# Autodesk Inventor assembly: Hanging Corner Cupboard (concept)
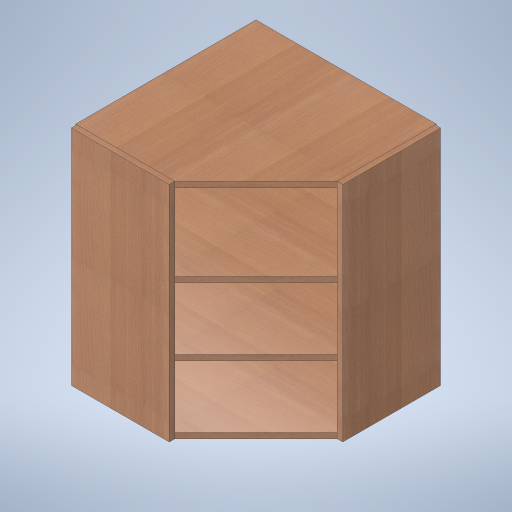
[picture p0: Inventor's stored thumbnail of the model, 512x512]
Saved by Autodesk Inventor 2024 (Build 280153000, 153)
## iProperties
RuleStatus: InUse
Created: 2017-01-19
Part Number: Hanging Corner Cupboard (concept)
Document SubType Name: Assembly
Designer: SvetlanaB
Author: SvetlanaB
## Documents named in this file (16)
- C:\W4INV 2024 Design\iBOX LIBRARY\Kitchen\Wall Cabinets\Corner Cupboard\Corner Cupboard.iam
- C:\W4INV 2024 Design\iBOX LIBRARY\Kitchen\Wall Cabinets\Corner Cupboard\Top.ipt
- C:\W4INV 2024 Design\iBOX LIBRARY\Kitchen\Wall Cabinets\Corner Cupboard\Right_side.ipt
- C:\W4INV 2024 Design\iBOX LIBRARY\Kitchen\Wall Cabinets\Corner Cupboard\Left_side.ipt
- C:\W4INV 2024 Design\iBOX LIBRARY\Kitchen\Wall Cabinets\Corner Cupboard\Back_panel.ipt
- C:\W4INV 2024 Design\iBOX LIBRARY\Kitchen\Wall Cabinets\Corner Cupboard\Back_left_panel.ipt
- C:\W4INV 2024 Design\iBOX LIBRARY\Kitchen\Wall Cabinets\Corner Cupboard\Back_right_panel.ipt
- C:\W4INV 2024 Design\_LIBRARY\Fixed joints\Minifix joint\MINIFIX D15 v2\Minifix D15 & Dowel L34 & Cap D15 PB T18 LH.ipt
- C:\W4INV 2024 Design\_LIBRARY\Fixed joints\Minifix joint\MINIFIX D15 v2\Minifix D15 & Dowel L34 & Cap D15 PB T18 RH.ipt
- C:\W4INV 2024 Design\iBOX LIBRARY\Kitchen\Wall Cabinets\Corner Cupboard\Cupboard (concept).ipt
- C:\W4INV 2024 Design\iBOX LIBRARY\Kitchen\Wall Cabinets\Corner Cupboard\Shelf.ipt
- C:\W4INV 2024 Design\_LIBRARY\Holders\Shelf holder D5\Shelf support D5 L16 with hole covers.ipt
- C:\W4INV 2024 Design\iBOX LIBRARY\Kitchen\Wall Cabinets\Corner Cupboard\Bottom.ipt
- C:\W4INV 2024 Design\_LIBRARY\Fixed joints\Minifix joint\MINIFIX D15 v2\Minifix D15 & Dowel L34 & Cap D15 PB T18 BT.ipt
- C:\W4INV 2023 Design\LIBRARY\Fixed joints\Minifix joint\MINIFIX D15 v2.ipt
- C:\W4INV 2023 Design\LIBRARY\Holders\Shelf holder D5.ipt
## Components (30 placed, 13 different names)
1. @Skeleton
2. Top:1 — Pillar Board Side Plane :1, Pillar Board Side Plane :2, Pillar Board Side Plane :5, Pillar Board Side Plane :6, Nestled Board Plane:9
3. Right_side:1 — Flush:2, Flush:4, Nestled Board Plane:5, Nestled Board Plane:6, Nestled Board Plane:7, Nestled Board Plane:8, Side Board Plane:3, Side Board Plane:4
4. Left_side:1 — Flush:1, Flush:3, Nestled Board Plane:1, Nestled Board Plane:2, Nestled Board Plane:3, Nestled Board Plane:4, Side Board Plane:1, Side Board Plane:2
5. Back_panel:1 — Pillar Board Side Plane :9, Pillar Board Side Plane :10, Side Board Plane:5
6. Back_left_panel:1
7. Back_right_panel:1
8. Minifix D15 & Dowel L34 & Cap D15 PB T18 RH:1 — Axis Plane:1, Nestled Board Plane:1, Pillar Board Side Plane :1
9. Minifix D15 & Dowel L34 & Cap D15 PB T18 LH:2 — Axis Plane:2, Nestled Board Plane:2, Pillar Board Side Plane :2
10. Minifix D15 & Dowel L34 & Cap D15 PB T18 LH:3 — Axis Plane:3, Nestled Board Plane:3, Axis Plane:11, Axis Plane:12, Axis Plane:13, Pillar Board Side Plane :3
11. Minifix D15 & Dowel L34 & Cap D15 PB T18 RH:4 — Axis Plane:4, Nestled Board Plane:4, Axis Plane:14, Pillar Board Side Plane :4
12. Minifix D15 & Dowel L34 & Cap D15 PB T18 LH:5 — Axis Plane:5, Nestled Board Plane:5, Pillar Board Side Plane :5
13. Minifix D15 & Dowel L34 & Cap D15 PB T18 RH:6 — Axis Plane:6, Nestled Board Plane:6, Pillar Board Side Plane :6
14. Minifix D15 & Dowel L34 & Cap D15 PB T18 RH:7 — Axis Plane:7, Nestled Board Plane:7, Pillar Board Side Plane :7
15. Minifix D15 & Dowel L34 & Cap D15 PB T18 LH:8 — Axis Plane:8, Nestled Board Plane:8, Pillar Board Side Plane :8
16. Minifix D15 & Dowel L34 & Cap D15 PB T18 BT:9 — Nestled Board Plane:9, Pillar Board Side Plane :9, Axis Plane:9
17. Minifix D15 & Dowel L34 & Cap D15 PB T18 BT:10 — Pillar Board Side Plane :10, Axis Plane:10, Axis Plane:15, Axis Plane:16, Nestled Board Plane:10
18. Bottom:1 — Nestled Board Plane:10, Pillar Board Side Plane :3, Pillar Board Side Plane :4, Pillar Board Side Plane :7, Pillar Board Side Plane :8
19. Shelf:1 — Shelf Pottom Plane:1, Shelf Pottom Plane:2, Shelf Pottom Plane:3, Shelf Pottom Plane:4, Shelf Pottom Plane:5
20. Shelf support D5 L16 with hole covers:2 — Axis Plane:18, Side Board Plane:2, Shelf Pottom Plane:2
21. Shelf support D5 L16 with hole covers:1 — Axis Plane:17, Side Board Plane:1, Shelf Pottom Plane:1
22. Shelf support D5 L16 with hole covers:5 — Side Board Plane:5, Shelf Pottom Plane:5, Axis Plane:21
23. Shelf support D5 L16 with hole covers:3 — Axis Plane:19, Side Board Plane:3, Shelf Pottom Plane:3
24. Shelf support D5 L16 with hole covers:4 — Axis Plane:20, Side Board Plane:4, Shelf Pottom Plane:4
25. Shelf:2
26. Shelf support D5 L16 with hole covers:6
27. Shelf support D5 L16 with hole covers:7
28. Shelf support D5 L16 with hole covers:8
29. Shelf support D5 L16 with hole covers:9
30. Shelf support D5 L16 with hole covers:10
## Component patterns: (2 elements, first: Shelf:1 + Shelf support D5 L16 with hole covers:2 + Shelf support D5 L16 with hole covers:1 + Shelf support D5 L16 with hole covers:5 + Shelf support D5 L16 with hole covers:3 + Shelf support D5 L16 with hole covers:4)
## Relationships (55: Mate 41, Flush 14)
- Flush:1 (-75 mm): Left_side:1
- Flush:2 (-75 mm): Right_side:1
- Flush:3 (-75 mm): Left_side:1
- Flush:4 (-75 mm): Right_side:1
- Axis Plane:1 [Mate]: Minifix D15 & Dowel L34 & Cap D15 PB T18 RH:1
- Nestled Board Plane:1 [Mate]: Left_side:1 ↔ Minifix D15 & Dowel L34 & Cap D15 PB T18 RH:1
- Pillar Board Side Plane :1 [Flush] (18 mm): Top:1 ↔ Minifix D15 & Dowel L34 & Cap D15 PB T18 RH:1
- Axis Plane:2 [Mate]: Minifix D15 & Dowel L34 & Cap D15 PB T18 LH:2
- Nestled Board Plane:2 [Mate]: Left_side:1 ↔ Minifix D15 & Dowel L34 & Cap D15 PB T18 LH:2
- Pillar Board Side Plane :2 [Flush] (18 mm): Top:1 ↔ Minifix D15 & Dowel L34 & Cap D15 PB T18 LH:2
- Axis Plane:3 [Mate]: Minifix D15 & Dowel L34 & Cap D15 PB T18 LH:3
- Nestled Board Plane:3 [Mate]: Left_side:1 ↔ Minifix D15 & Dowel L34 & Cap D15 PB T18 LH:3
- Axis Plane:4 [Mate]: Minifix D15 & Dowel L34 & Cap D15 PB T18 RH:4
- Nestled Board Plane:4 [Mate]: Left_side:1 ↔ Minifix D15 & Dowel L34 & Cap D15 PB T18 RH:4
- Axis Plane:5 [Mate]: Minifix D15 & Dowel L34 & Cap D15 PB T18 LH:5
- Nestled Board Plane:5 [Mate]: Right_side:1 ↔ Minifix D15 & Dowel L34 & Cap D15 PB T18 LH:5
- Pillar Board Side Plane :5 [Flush] (18 mm): Top:1 ↔ Minifix D15 & Dowel L34 & Cap D15 PB T18 LH:5
- Axis Plane:6 [Mate]: Minifix D15 & Dowel L34 & Cap D15 PB T18 RH:6
- Nestled Board Plane:6 [Mate]: Right_side:1 ↔ Minifix D15 & Dowel L34 & Cap D15 PB T18 RH:6
- Pillar Board Side Plane :6 [Flush] (18 mm): Top:1 ↔ Minifix D15 & Dowel L34 & Cap D15 PB T18 RH:6
- Axis Plane:7 [Mate]: Minifix D15 & Dowel L34 & Cap D15 PB T18 RH:7
- Nestled Board Plane:7 [Mate]: Right_side:1 ↔ Minifix D15 & Dowel L34 & Cap D15 PB T18 RH:7
- Axis Plane:8 [Mate]: Minifix D15 & Dowel L34 & Cap D15 PB T18 LH:8
- Nestled Board Plane:8 [Mate]: Right_side:1 ↔ Minifix D15 & Dowel L34 & Cap D15 PB T18 LH:8
- Nestled Board Plane:9 [Mate]: Top:1 ↔ Minifix D15 & Dowel L34 & Cap D15 PB T18 BT:9
- Pillar Board Side Plane :9 [Flush] (18 mm): Back_panel:1 ↔ Minifix D15 & Dowel L34 & Cap D15 PB T18 BT:9
- Axis Plane:9 [Mate]: Minifix D15 & Dowel L34 & Cap D15 PB T18 BT:9
- Pillar Board Side Plane :10 [Flush] (18 mm): Back_panel:1 ↔ Minifix D15 & Dowel L34 & Cap D15 PB T18 BT:10
- Axis Plane:10 [Mate]: Minifix D15 & Dowel L34 & Cap D15 PB T18 BT:10
- Axis Plane:11 [Mate]: Minifix D15 & Dowel L34 & Cap D15 PB T18 LH:3
- Axis Plane:12 [Mate]: Minifix D15 & Dowel L34 & Cap D15 PB T18 LH:3
- Axis Plane:13 [Mate]: Minifix D15 & Dowel L34 & Cap D15 PB T18 LH:3
- Axis Plane:14 [Mate]: Minifix D15 & Dowel L34 & Cap D15 PB T18 RH:4
- Axis Plane:15 [Mate]: Minifix D15 & Dowel L34 & Cap D15 PB T18 BT:10
- Axis Plane:16 [Mate]: Minifix D15 & Dowel L34 & Cap D15 PB T18 BT:10
- Axis Plane:17 [Mate]: Shelf support D5 L16 with hole covers:1
- Side Board Plane:1 [Mate]: Left_side:1 ↔ Shelf support D5 L16 with hole covers:1
- Shelf Pottom Plane:1 [Mate] (2.5 mm): Shelf:1 ↔ Shelf support D5 L16 with hole covers:1
- Axis Plane:18 [Mate]: Shelf support D5 L16 with hole covers:2
- Side Board Plane:2 [Mate]: Left_side:1 ↔ Shelf support D5 L16 with hole covers:2
- Shelf Pottom Plane:2 [Mate] (2.5 mm): Shelf:1 ↔ Shelf support D5 L16 with hole covers:2
- Axis Plane:19 [Mate]: Shelf support D5 L16 with hole covers:3
- Side Board Plane:3 [Mate]: Right_side:1 ↔ Shelf support D5 L16 with hole covers:3
- Shelf Pottom Plane:3 [Mate] (2.5 mm): Shelf:1 ↔ Shelf support D5 L16 with hole covers:3
- Axis Plane:20 [Mate]: Shelf support D5 L16 with hole covers:4
- Side Board Plane:4 [Mate]: Right_side:1 ↔ Shelf support D5 L16 with hole covers:4
- Shelf Pottom Plane:4 [Mate] (2.5 mm): Shelf:1 ↔ Shelf support D5 L16 with hole covers:4
- Side Board Plane:5 [Mate]: Back_panel:1 ↔ Shelf support D5 L16 with hole covers:5
- Shelf Pottom Plane:5 [Mate] (2.5 mm): Shelf:1 ↔ Shelf support D5 L16 with hole covers:5
- Axis Plane:21 [Mate]: Shelf support D5 L16 with hole covers:5
- Nestled Board Plane:10 [Mate]: Minifix D15 & Dowel L34 & Cap D15 PB T18 BT:10 ↔ Bottom:1
- Pillar Board Side Plane :3 [Flush] (18 mm): Minifix D15 & Dowel L34 & Cap D15 PB T18 LH:3 ↔ Bottom:1
- Pillar Board Side Plane :4 [Flush] (18 mm): Minifix D15 & Dowel L34 & Cap D15 PB T18 RH:4 ↔ Bottom:1
- Pillar Board Side Plane :7 [Flush] (18 mm): Minifix D15 & Dowel L34 & Cap D15 PB T18 RH:7 ↔ Bottom:1
- Pillar Board Side Plane :8 [Flush] (18 mm): Minifix D15 & Dowel L34 & Cap D15 PB T18 LH:8 ↔ Bottom:1
## Named parameters: Panel_thickness = 18 mm, Right_cupboard_side = 320 mm, Left_cupboard_side = 320 mm, Shelf_number = 2, Shelf_space_from_bottom = 200 mm, Space_between_shelfs = 200 mm
